# Autodesk Inventor assembly: bloc_double106
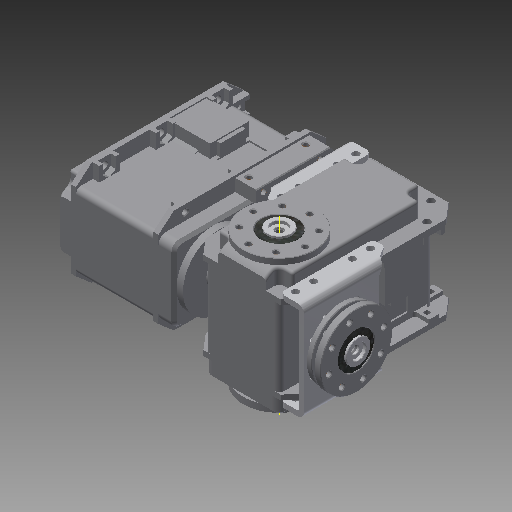
[picture p0: Inventor's stored thumbnail of the model, 512x512]
Saved by Autodesk Inventor 2018 (Build 220112000, 112)
## iProperties
Created: 2017-02-17
Part Number: bloc_double106
Document SubType Name: Assembly
Designer: steve
Mass: 340.305 g
Surface Area: 512.023 cm^2
Volume: 186.598 cm^3
Density: 1.82373 g/cm^3
Author: steve
## Documents named in this file (8)
- C:\Users\medrimonia\Dropbox\SigmaBan\SigmaBanV2.1\bloc_double106.iam
- C:\Users\medrimonia\Dropbox\SigmaBan\SigmaBanV2.1\MX-106T.ipt
- C:\Users\medrimonia\Dropbox\SigmaBan\SigmaBanV2.1\RX64-CAP.ipt
- C:\Users\medrimonia\Dropbox\SigmaBan\SigmaBanV2.1\dynamixel\horn\HN05-i101.ipt
- C:\Users\medrimonia\Dropbox\SigmaBan\SigmaBanV2.1\MF128ZZ.ipt
- C:\Users\medrimonia\Dropbox\SigmaBan\SigmaBanV2.1\dynamixel\frames\FR08-B101.ipt
- C:\Users\medrimonia\Dropbox\SigmaBan\SigmaBanV2.1\FR05-S101.ipt
- C:\Users\medrimonia\Dropbox\SigmaBan\SigmaBanV2.1\dynamixel\frames\FR05-F101.ipt
## Components (13 placed, 7 different names)
1. MX-106T:1 — Mate:8, Mate:26, Mate:27, Mate:30, Flush:1, Mate:39, Mate:40, Mate:41, Mate:43, Mate:44, Mate:45
2. MX-106T:2 — Mate:13, Mate:31, Mate:35, Mate:36, Mate:37, Mate:56, Mate:57
3. HN05-i101:2 — Mate:55, Mate:56
4. RX64-CAP:1 — Mate:26
5. HN05-i101:1 — Flush:1
6. MF128ZZ:1 — Mate:27
7. FR08-B101:1 — Mate:35, Mate:36, Mate:37, Mate:46, Mate:47
8. FR05-S101:1 — Mate:39, Mate:40, Mate:41, Mate:48, Mate:53
9. FR05-S101:2 — Mate:43, Mate:44, Mate:45, Mate:46, Mate:47
10. FR05-F101:1 — Mate:48, Mate:51, Mate:52, Mate:53
11. RX64-CAP:2 — Mate:51, Mate:52, Mate:54
12. MF128ZZ:2 — Mate:54, Mate:55, Mate:57
13. MF128ZZ:3
## Relationships (29: Mate 28, Flush 1)
- Mate:8: MX-106T:1
- Mate:13: MX-106T:2
- [Mate]: HN05-i101:1 ↔ MF128ZZ:1
- [Mate]: RX64-CAP:1 ↔ MF128ZZ:1
- [Mate]: RX64-CAP:1 ↔ MF128ZZ:1
- Mate:26: MX-106T:1 ↔ RX64-CAP:1
- Mate:27: MX-106T:1 ↔ MF128ZZ:1
- Mate:30: MX-106T:1
- Mate:31: MX-106T:2
- Flush:1 (-3 mm): MX-106T:1 ↔ HN05-i101:1
- Mate:35: MX-106T:2 ↔ FR08-B101:1
- Mate:36: MX-106T:2 ↔ FR08-B101:1
- Mate:37: MX-106T:2 ↔ FR08-B101:1
- Mate:39: MX-106T:1 ↔ FR05-S101:1
- Mate:40: MX-106T:1 ↔ FR05-S101:1
- Mate:41: MX-106T:1 ↔ FR05-S101:1
- Mate:43: MX-106T:1 ↔ FR05-S101:2
- Mate:44: MX-106T:1 ↔ FR05-S101:2
- Mate:45: MX-106T:1 ↔ FR05-S101:2
- Mate:46: FR08-B101:1 ↔ FR05-S101:2
- Mate:47: FR08-B101:1 ↔ FR05-S101:2
- Mate:48: FR05-S101:1 ↔ FR05-F101:1
- Mate:51: FR05-F101:1 ↔ RX64-CAP:2
- Mate:52: FR05-F101:1 ↔ RX64-CAP:2
- Mate:53: FR05-S101:1 ↔ FR05-F101:1
- Mate:54: RX64-CAP:2 ↔ MF128ZZ:2
- Mate:55: HN05-i101:2 ↔ MF128ZZ:2
- Mate:56: MX-106T:2 ↔ HN05-i101:2
- Mate:57: MX-106T:2 ↔ MF128ZZ:2
## Named parameters: d28_d26 = 0 mm, d29_d27 = 0 mm
